# Autodesk Inventor assembly: Test_Rig_Assembly
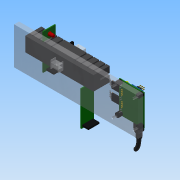
[picture p0: Inventor's stored thumbnail of the model, 180x180]
Saved by Autodesk Inventor 2016 (Build 200138000, 138)
## iProperties
Created: 2015-05-19
Part Number: Test_Rig_Assembly
Document SubType Name: Assembly
Designer: Openlab
Author: Openlab
## Documents named in this file (9)
- D:\Alexey\HS-Spectrophotometer\parts\Test\Assembly.iam
- D:\Alexey\HS-Spectrophotometer\parts\Test\Distance_test_rig.ipt
- D:\Alexey\HS-Spectrophotometer\parts\Test\LED_board.ipt
- D:\Alexey\HS-Spectrophotometer\parts\Test\Sensor_board.ipt
- D:\Alexey\HS-Spectrophotometer\parts\Test\Base.ipt
- D:\Alexey\HS-Spectrophotometer\parts\Common\Microcontroller_board_Nano_square.iam
- D:\Alexey\HS-Spectrophotometer\parts\Common\Support_washer.ipt
- D:\Alexey\HS-Spectrophotometer\parts\Common\Cuvette.ipt
- D:\Alexey\HS-Spectrophotometer\parts\Test\PCB_slit_circle_1.5mm.ipt
## Components (11 placed, 8 different names)
1. Distance_test_rig:1 — Mate:1, Mate:2, Mate:3, Mate:4, Mate:5, Flush:1, Flush:2, Mate:19, Mate:20, Mate:21, Mate:22, Mate:23, Mate:24
2. LED_board:1 — Mate:1, Mate:2
3. Sensor_board:1 — Mate:3, Mate:4
4. Base:1 — Mate:5, Flush:1, Flush:2, Mate:6, Mate:7, Mate:8, Mate:9, Mate:10, Mate:11, Mate:12, Mate:13
5. Microcontroller_board_Nano_square:1 [sub-assembly] — Mate:14, Mate:15, Mate:16
6. Support_washer:1 — Mate:9, Mate:13, Mate:15
7. Support_washer:2 — Mate:8, Mate:12
8. Support_washer:3 — Mate:6, Mate:10, Mate:14, Mate:16
9. Support_washer:4 — Mate:7, Mate:11
10. Cuvette:1 — Mate:19, Mate:20, Mate:21
11. PCB_slit_circle_1.5mm:1 — Mate:22, Mate:23, Mate:24
## Relationships (24: Mate 22, Flush 2)
- Mate:1: Distance_test_rig:1 ↔ LED_board:1
- Mate:2: Distance_test_rig:1 ↔ LED_board:1
- Mate:3: Distance_test_rig:1 ↔ Sensor_board:1
- Mate:4: Distance_test_rig:1 ↔ Sensor_board:1
- Mate:5: Distance_test_rig:1 ↔ Base:1
- Flush:1 (10 mm): Distance_test_rig:1 ↔ Base:1
- Flush:2 (-15 mm): Distance_test_rig:1 ↔ Base:1
- Mate:6: Base:1 ↔ Support_washer:3
- Mate:7: Base:1 ↔ Support_washer:4
- Mate:8: Base:1 ↔ Support_washer:2
- Mate:9: Base:1 ↔ Support_washer:1
- Mate:10: Base:1 ↔ Support_washer:3
- Mate:11: Base:1 ↔ Support_washer:4
- Mate:12: Base:1 ↔ Support_washer:2
- Mate:13: Base:1 ↔ Support_washer:1
- Mate:14: Microcontroller_board_Nano_square:1 ↔ Support_washer:3
- Mate:15: Microcontroller_board_Nano_square:1 ↔ Support_washer:1
- Mate:16: Microcontroller_board_Nano_square:1 ↔ Support_washer:3
- Mate:19: Distance_test_rig:1 ↔ Cuvette:1
- Mate:20: Distance_test_rig:1 ↔ Cuvette:1
- Mate:21: Distance_test_rig:1 ↔ Cuvette:1
- Mate:22: Distance_test_rig:1 ↔ PCB_slit_circle_1.5mm:1
- Mate:23: Distance_test_rig:1 ↔ PCB_slit_circle_1.5mm:1
- Mate:24: Distance_test_rig:1 ↔ PCB_slit_circle_1.5mm:1
